# Autodesk Inventor assembly: PotentiometerAssembly
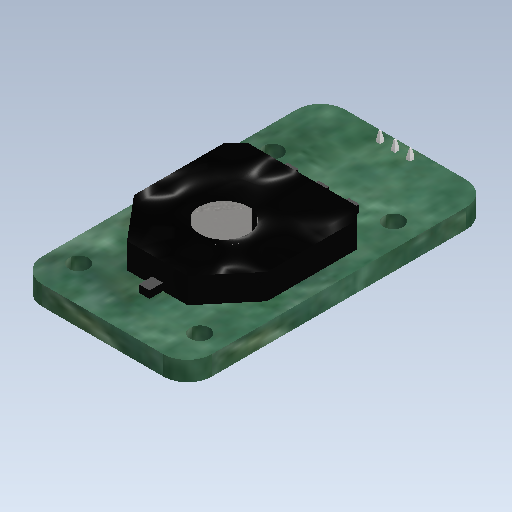
[picture p0: Inventor's stored thumbnail of the model, 512x512]
Saved by Autodesk Inventor 2020 (Build 240168000, 168)
## iProperties
Created: 2020-01-18
Part Number: PotentiometerAssembly
Document SubType Name: Assembly
Designer: sami_
Author: sami_
## Documents named in this file (5)
- C:\Users\sami_\Documents\V1.5\Workgroups\NotInProject\PINKY\PotentiometerAssembly.iam
- C:\Users\sami_\Documents\V1.5\Workgroups\NotInProject\PINKY\potentiometerbody.ipt
- C:\Users\sami_\Documents\V1.5\Workgroups\NotInProject\PINKY\potentiometerspinny.ipt
- C:\Users\sami_\Documents\V1.5\Workgroups\NotInProject\PINKY\potentiometerpcb.ipt
- C:\Users\sami_\Documents\V1.5\Workgroups\NotInProject\connector.ipt
## Components (4 placed, 4 different names)
1. potentiometerbody:1 — Rotational:1, Rigid:1
2. potentiometerspinny:1 — Rotational:1
3. potentiometerpcb:1 — Rigid:1, Rigid:2
4. connector:1 — Rigid:2
## Relationships (3: WeldJoint 2, RevoluteJoint 1)
- Rotational:1 [RevoluteJoint] (0.02 mm): potentiometerbody:1 ↔ potentiometerspinny:1
- Rigid:1 [WeldJoint]: potentiometerbody:1 ↔ potentiometerpcb:1
- Rigid:2 [WeldJoint]: potentiometerpcb:1 ↔ connector:1
